# Autodesk Inventor assembly: eboard
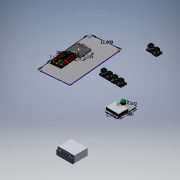
[picture p0: Inventor's stored thumbnail of the model, 180x180]
Saved by Autodesk Inventor 2016 (Build 200138000, 138)
## iProperties
Created: 2016-01-21
Part Number: eboard
Document SubType Name: Assembly
Designer: Administrator
Author: Administrator
## Documents named in this file (9)
- C:\Users\Administrator\Desktop\3192CAD\InitialRobotProto\eboard.iam
- C:\Users\Administrator\Desktop\3192CAD\InitialRobotProto\eboardbaseplate.ipt
- C:\Users\Administrator\Desktop\3192CAD\InitialRobotProto\CS_Controller_ROBORIO.ipt
- C:\Users\Administrator\Desktop\3192CAD\InitialRobotProto\CS_DistrPanel_14-806880.ipt
- C:\Users\Administrator\Desktop\3192CAD\InitialRobotProto\CS_Controller_217-2769.ipt
- C:\Users\Administrator\Desktop\3192CAD\InitialRobotProto\fc16-036_Battery.iam
- C:\Users\Administrator\Desktop\3192CAD\InitialRobotProto\ELEC_SignalLED_855PB-B12ME522.ipt
- C:\Users\Administrator\Desktop\3192CAD\InitialRobotProto\CS_WirelessBridge_DAP1522.ipt
- C:\Users\Administrator\Desktop\3192CAD\InitialRobotProto\eboardpartisland.ipt
## Components (13 placed, 8 different names)
1. eboardbaseplate:1 — Mate:1, Mate:2, Mate:3, Mate:4, Mate:5, Mate:6, Mate:7, Mate:8, Mate:9, Mate:10, Mate:11, Mate:12
2. CS_Controller_ROBORIO:1 — Mate:1, Mate:11, Mate:12
3. CS_DistrPanel_14-806880:1 — Mate:2, Mate:9, Mate:10
4. CS_Controller_217-2769:1 — Mate:3
5. CS_Controller_217-2769:2 — Mate:6
6. CS_Controller_217-2769:3 — Mate:7
7. CS_Controller_217-2769:4 — Mate:8
8. CS_Controller_217-2769:5 — Mate:5
9. CS_Controller_217-2769:6 — Mate:4
10. fc16-036_Battery:1 [sub-assembly]
11. ELEC_SignalLED_855PB-B12ME522:1 — Mate:13, Mate:14
12. CS_WirelessBridge_DAP1522:1 — Mate:15
13. eboardpartisland:1 — Mate:13, Mate:14, Mate:15
## Relationships (15: Mate 15)
- Mate:1: eboardbaseplate:1 ↔ CS_Controller_ROBORIO:1
- Mate:2: eboardbaseplate:1 ↔ CS_DistrPanel_14-806880:1
- Mate:3: eboardbaseplate:1 ↔ CS_Controller_217-2769:1
- Mate:4: eboardbaseplate:1 ↔ CS_Controller_217-2769:6
- Mate:5: eboardbaseplate:1 ↔ CS_Controller_217-2769:5
- Mate:6: eboardbaseplate:1 ↔ CS_Controller_217-2769:2
- Mate:7: eboardbaseplate:1 ↔ CS_Controller_217-2769:3
- Mate:8: eboardbaseplate:1 ↔ CS_Controller_217-2769:4
- Mate:9: eboardbaseplate:1 ↔ CS_DistrPanel_14-806880:1
- Mate:10: eboardbaseplate:1 ↔ CS_DistrPanel_14-806880:1
- Mate:11: eboardbaseplate:1 ↔ CS_Controller_ROBORIO:1
- Mate:12: eboardbaseplate:1 ↔ CS_Controller_ROBORIO:1
- Mate:13: ELEC_SignalLED_855PB-B12ME522:1 ↔ eboardpartisland:1
- Mate:14: ELEC_SignalLED_855PB-B12ME522:1 ↔ eboardpartisland:1
- Mate:15: CS_WirelessBridge_DAP1522:1 ↔ eboardpartisland:1
